# Autodesk Inventor assembly: A2017_T3_06
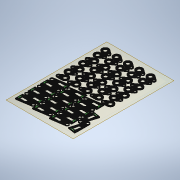
[picture p0: Inventor's stored thumbnail of the model, 180x180]
Saved by Autodesk Inventor 2022 (Build 260153000, 153)
## iProperties
Created: 2022-09-28
Part Number: A2017_T3_06
Document SubType Name: Assembly
Designer: Masato
Author: Masato
## Documents named in this file (4)
- C:\Users\6343y\ドキュメント\Inventor\SUSTAINA-OP\Cam\A2017_T3\A2017_T3_06.iam
- C:\Users\6343y\ドキュメント\Inventor\SUSTAINA-OP\Cam\DisposableBoard.ipt
- C:\Users\6343y\ドキュメント\Inventor\SUSTAINA-OP\LowerBody\Leg_joint\Leg_joint_slider_frame.ipt
- C:\Users\6343y\ドキュメント\Inventor\SUSTAINA-OP\LowerBody\Slider_crank\Slider_crank_horn.ipt
## Components (56 placed, 3 different names)
1. DisposableBoard:1 — フラッシュ:1, フラッシュ:2, フラッシュ:3, フラッシュ:4, フラッシュ:5, フラッシュ:6, 正接:1, フラッシュ:7, 正接:2, メイト:5, 正接:5, 正接:6, 正接:7
2. Leg_joint_slider_frame:2 — メイト:1, メイト:3, 正接:1
3. Leg_joint_slider_frame:1 — メイト:2, メイト:3, フラッシュ:5, フラッシュ:6
4. Leg_joint_slider_frame:3
5. Leg_joint_slider_frame:4
6. Leg_joint_slider_frame:5
7. Leg_joint_slider_frame:6
8. Leg_joint_slider_frame:7
9. Leg_joint_slider_frame:8
10. Leg_joint_slider_frame:9
11. Leg_joint_slider_frame:10
12. Leg_joint_slider_frame:11 — メイト:7
13. Leg_joint_slider_frame:12
14. Leg_joint_slider_frame:13 — メイト:10
15. Leg_joint_slider_frame:14
16. Leg_joint_slider_frame:15
17. Leg_joint_slider_frame:16
18. Leg_joint_slider_frame:17
19. Leg_joint_slider_frame:18
20. Leg_joint_slider_frame:43 — メイト:4, フラッシュ:7, 正接:2, メイト:6
21. Leg_joint_slider_frame:44 — メイト:5, メイト:6, メイト:7
22. Slider_crank_horn:2 — メイト:9, メイト:11, 正接:6
23. Slider_crank_horn:1 — メイト:8, メイト:10, 正接:5, メイト:11
24. Slider_crank_horn:3
25. Slider_crank_horn:4
26. Slider_crank_horn:5 — メイト:13
27. Slider_crank_horn:6
28. Slider_crank_horn:7
29. Slider_crank_horn:8
30. Slider_crank_horn:9
31. Slider_crank_horn:10
32. Slider_crank_horn:11
33. Slider_crank_horn:12
34. Slider_crank_horn:13
35. Slider_crank_horn:14
36. Slider_crank_horn:15
37. Slider_crank_horn:16
38. Slider_crank_horn:17
39. Slider_crank_horn:18
40. Slider_crank_horn:19
41. Slider_crank_horn:20
42. Slider_crank_horn:21
43. Slider_crank_horn:22
44. Slider_crank_horn:23
45. Slider_crank_horn:24
46. Slider_crank_horn:25
47. Slider_crank_horn:26
48. Slider_crank_horn:27
49. Slider_crank_horn:28
50. Slider_crank_horn:29
51. Slider_crank_horn:30
52. Slider_crank_horn:31 — メイト:12, メイト:13, 正接:7
53. Slider_crank_horn:32
54. Slider_crank_horn:33
55. Slider_crank_horn:34
56. Slider_crank_horn:35
## Component patterns: (9 elements, first: Leg_joint_slider_frame:2 + Leg_joint_slider_frame:1), (1 elements, first: Leg_joint_slider_frame:43 + Leg_joint_slider_frame:44), (15 elements, first: Slider_crank_horn:2 + Slider_crank_horn:1), (5 elements, first: Slider_crank_horn:31)
## Relationships (25: Mate 13, Flush 7, Tangent 5)
- フラッシュ:1 [Flush]: DisposableBoard:1
- フラッシュ:2 [Flush]: DisposableBoard:1
- フラッシュ:3 [Flush]: DisposableBoard:1
- フラッシュ:4 [Flush]: DisposableBoard:1
- メイト:1 [Mate]: Leg_joint_slider_frame:2
- メイト:2 [Mate]: Leg_joint_slider_frame:1
- メイト:3 [Mate] (2.1 mm): Leg_joint_slider_frame:2 ↔ Leg_joint_slider_frame:1
- フラッシュ:5 [Flush] (2.1 mm): DisposableBoard:1 ↔ Leg_joint_slider_frame:1
- フラッシュ:6 [Flush] (2.1 mm): DisposableBoard:1 ↔ Leg_joint_slider_frame:1
- 正接:1 [Tangent] (2.1 mm): DisposableBoard:1 ↔ Leg_joint_slider_frame:2
- メイト:4 [Mate]: Leg_joint_slider_frame:43
- フラッシュ:7 [Flush] (2.1 mm): DisposableBoard:1 ↔ Leg_joint_slider_frame:43
- 正接:2 [Tangent] (3.5 mm): DisposableBoard:1 ↔ Leg_joint_slider_frame:43
- メイト:5 [Mate]: DisposableBoard:1 ↔ Leg_joint_slider_frame:44
- メイト:6 [Mate] (2.1 mm): Leg_joint_slider_frame:43 ↔ Leg_joint_slider_frame:44
- メイト:7 [Mate] (2.1 mm): Leg_joint_slider_frame:11 ↔ Leg_joint_slider_frame:44
- メイト:8 [Mate]: Slider_crank_horn:1
- メイト:9 [Mate]: Slider_crank_horn:2
- メイト:10 [Mate] (2.1 mm): Leg_joint_slider_frame:13 ↔ Slider_crank_horn:1
- 正接:5 [Tangent] (2.1 mm): DisposableBoard:1 ↔ Slider_crank_horn:1
- メイト:11 [Mate] (2.1 mm): Slider_crank_horn:2 ↔ Slider_crank_horn:1
- 正接:6 [Tangent] (2.1 mm): DisposableBoard:1 ↔ Slider_crank_horn:2
- メイト:12 [Mate]: Slider_crank_horn:31
- メイト:13 [Mate] (2.1 mm): Slider_crank_horn:5 ↔ Slider_crank_horn:31
- 正接:7 [Tangent] (2.1 mm): DisposableBoard:1 ↔ Slider_crank_horn:31
